# Autodesk Inventor assembly: Rubik's Chassis
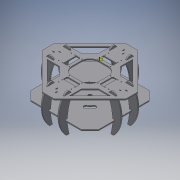
[picture p0: Inventor's stored thumbnail of the model, 180x180]
Saved by Autodesk Inventor 2017 (Build 210142000, 142)
## iProperties
Created: 2018-12-09
Part Number: Rubik's Chassis
Document SubType Name: Assembly
Designer: Eric the Great
Author: Eric the Great
## Documents named in this file (4)
- C:\Users\Eric the Great\Documents\Cornell University\ECE 5725\Final Project\Rubik's Chassis.iam
- C:\Users\Eric the Great\Documents\Cornell University\ECE 5725\Final Project\CAD\Base Plate.ipt
- C:\Users\Eric the Great\Documents\Cornell University\ECE 5725\Final Project\CAD\bottom plate.ipt
- C:\Users\Eric the Great\Documents\Cornell University\ECE 5725\Final Project\CAD\leg.ipt
## Components (10 placed, 3 different names)
1. Base Plate:1 — Mate:2, Mate:5, Mate:6
2. bottom plate:1 — Mate:2, Mate:3, Mate:4
3. leg:1 — Flush:1, Flush:2, Mate:1
4. leg:2 — Flush:1, Flush:2, Mate:1, Mate:3, Mate:4, Mate:5, Mate:6
5. leg:3
6. leg:4
7. leg:5
8. leg:6
9. leg:7
10. leg:8
## Component patterns: (4 elements, first: leg:1 + leg:2)
## Relationships (8: Mate 6, Flush 2)
- Flush:1: leg:1 ↔ leg:2
- Flush:2: leg:1 ↔ leg:2
- Mate:1 (70 mm): leg:1 ↔ leg:2
- Mate:2: Base Plate:1 ↔ bottom plate:1
- Mate:3: bottom plate:1 ↔ leg:2
- Mate:4: bottom plate:1 ↔ leg:2
- Mate:5: Base Plate:1 ↔ leg:2
- Mate:6: Base Plate:1 ↔ leg:2
